# Autodesk Inventor assembly: Base-soporte
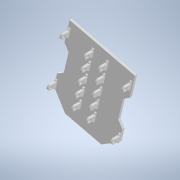
[picture p0: Inventor's stored thumbnail of the model, 180x180]
Saved by Autodesk Inventor 2021 (Build 250183000, 183)
## iProperties
Created: 2021-02-07
Part Number: Base-soporte
Document SubType Name: Assembly
Designer: rotje
Author: rotje
## Documents named in this file (5)
- C:\Users\rotje\Documents\Inventor\MSF\Base-soporte.iam
- C:\Users\rotje\Documents\Inventor\MSF\BaseCarro.ipt
- C:\Users\rotje\Documents\Inventor\MSF\sopoetellantas.ipt
- C:\Users\rotje\Documents\Inventor\MSF\soporte_para_engrane.ipt
- C:\Users\rotje\Documents\Inventor\MSF\din_912-m5x0_8-20-8_8.ipt
## Components (43 placed, 4 different names)
1. BaseCarro:1 — Insertar:1, Insertar:2, Insertar:3, Insertar:4, Insertar:5, Insertar:6, Insertar:7, Insertar:8, Insertar:9, Insertar:10, Insertar:11, Insertar:12, Insertar:13, Insertar:14, Insertar:15, Insertar:16, Insertar:17, Insertar:18, Insertar:19, Insertar:20, Insertar:21, Insertar:22, Insertar:23, Insertar:24, Insertar:25, Insertar:26, Insertar:27, Insertar:28
2. sopoetellantas:1 — Insertar:1, Insertar:2, Insertar:29, Insertar:30
3. sopoetellantas:2 — Insertar:7, Insertar:8, Insertar:35, Insertar:36
4. sopoetellantas:3 — Insertar:15, Insertar:16, Insertar:49, Insertar:50
5. sopoetellantas:4 — Insertar:9, Insertar:10, Insertar:51, Insertar:52
6. sopoetellantas:5 — Insertar:3, Insertar:4, Insertar:31, Insertar:32
7. sopoetellantas:6 — Insertar:5, Insertar:6, Insertar:33, Insertar:34
8. sopoetellantas:7 — Insertar:13, Insertar:14, Insertar:55, Insertar:56
9. sopoetellantas:8 — Insertar:11, Insertar:12, Insertar:53, Insertar:54
10. soporte_para_engrane:1 — Insertar:23, Insertar:24, Insertar:39, Insertar:40
11. soporte_para_engrane:2 — Insertar:25, Insertar:26, Insertar:41, Insertar:42
12. soporte_para_engrane:3 — Insertar:27, Insertar:28, Insertar:47, Insertar:48
13. soporte_para_engrane:4 — Insertar:17, Insertar:18, Insertar:37, Insertar:38
14. soporte_para_engrane:5 — Insertar:19, Insertar:20, Insertar:43, Insertar:44
15. soporte_para_engrane:6 — Insertar:21, Insertar:22, Insertar:45, Insertar:46
16. din_912-m5x0_8-20-8_8:1 — Insertar:29
17. din_912-m5x0_8-20-8_8:2 — Insertar:30
18. din_912-m5x0_8-20-8_8:3 — Insertar:32
19. din_912-m5x0_8-20-8_8:4 — Insertar:31
20. din_912-m5x0_8-20-8_8:5 — Insertar:33
21. din_912-m5x0_8-20-8_8:6 — Insertar:34
22. din_912-m5x0_8-20-8_8:7 — Insertar:35
23. din_912-m5x0_8-20-8_8:8 — Insertar:36
24. din_912-m5x0_8-20-8_8:9 — Insertar:39
25. din_912-m5x0_8-20-8_8:10 — Insertar:40
26. din_912-m5x0_8-20-8_8:11 — Insertar:41
27. din_912-m5x0_8-20-8_8:12 — Insertar:42
28. din_912-m5x0_8-20-8_8:13 — Insertar:47
29. din_912-m5x0_8-20-8_8:14 — Insertar:48
30. din_912-m5x0_8-20-8_8:15 — Insertar:49
31. din_912-m5x0_8-20-8_8:16 — Insertar:50
32. din_912-m5x0_8-20-8_8:17 — Insertar:53
33. din_912-m5x0_8-20-8_8:18 — Insertar:55
34. din_912-m5x0_8-20-8_8:19 — Insertar:54
35. din_912-m5x0_8-20-8_8:20 — Insertar:56
36. din_912-m5x0_8-20-8_8:21 — Insertar:51
37. din_912-m5x0_8-20-8_8:22 — Insertar:52
38. din_912-m5x0_8-20-8_8:23 — Insertar:37
39. din_912-m5x0_8-20-8_8:24 — Insertar:38
40. din_912-m5x0_8-20-8_8:25 — Insertar:43
41. din_912-m5x0_8-20-8_8:26 — Insertar:44
42. din_912-m5x0_8-20-8_8:27 — Insertar:45
43. din_912-m5x0_8-20-8_8:28 — Insertar:46
## Relationships (56: Insert 56)
- Insertar:1: BaseCarro:1 ↔ sopoetellantas:1
- Insertar:2: BaseCarro:1 ↔ sopoetellantas:1
- Insertar:3: BaseCarro:1 ↔ sopoetellantas:5
- Insertar:4: BaseCarro:1 ↔ sopoetellantas:5
- Insertar:5: BaseCarro:1 ↔ sopoetellantas:6
- Insertar:6: BaseCarro:1 ↔ sopoetellantas:6
- Insertar:7: BaseCarro:1 ↔ sopoetellantas:2
- Insertar:8: BaseCarro:1 ↔ sopoetellantas:2
- Insertar:9: BaseCarro:1 ↔ sopoetellantas:4
- Insertar:10: BaseCarro:1 ↔ sopoetellantas:4
- Insertar:11: BaseCarro:1 ↔ sopoetellantas:8
- Insertar:12: BaseCarro:1 ↔ sopoetellantas:8
- Insertar:13: BaseCarro:1 ↔ sopoetellantas:7
- Insertar:14: BaseCarro:1 ↔ sopoetellantas:7
- Insertar:15: BaseCarro:1 ↔ sopoetellantas:3
- Insertar:16: BaseCarro:1 ↔ sopoetellantas:3
- Insertar:17: BaseCarro:1 ↔ soporte_para_engrane:4
- Insertar:18: BaseCarro:1 ↔ soporte_para_engrane:4
- Insertar:19: BaseCarro:1 ↔ soporte_para_engrane:5
- Insertar:20: BaseCarro:1 ↔ soporte_para_engrane:5
- Insertar:21: BaseCarro:1 ↔ soporte_para_engrane:6
- Insertar:22: BaseCarro:1 ↔ soporte_para_engrane:6
- Insertar:23: BaseCarro:1 ↔ soporte_para_engrane:1
- Insertar:24: BaseCarro:1 ↔ soporte_para_engrane:1
- Insertar:25: BaseCarro:1 ↔ soporte_para_engrane:2
- Insertar:26: BaseCarro:1 ↔ soporte_para_engrane:2
- Insertar:27: BaseCarro:1 ↔ soporte_para_engrane:3
- Insertar:28: BaseCarro:1 ↔ soporte_para_engrane:3
- Insertar:29: sopoetellantas:1 ↔ din_912-m5x0_8-20-8_8:1
- Insertar:30: sopoetellantas:1 ↔ din_912-m5x0_8-20-8_8:2
- Insertar:31: sopoetellantas:5 ↔ din_912-m5x0_8-20-8_8:4
- Insertar:32: sopoetellantas:5 ↔ din_912-m5x0_8-20-8_8:3
- Insertar:33: sopoetellantas:6 ↔ din_912-m5x0_8-20-8_8:5
- Insertar:34: sopoetellantas:6 ↔ din_912-m5x0_8-20-8_8:6
- Insertar:35: sopoetellantas:2 ↔ din_912-m5x0_8-20-8_8:7
- Insertar:36: sopoetellantas:2 ↔ din_912-m5x0_8-20-8_8:8
- Insertar:37: soporte_para_engrane:4 ↔ din_912-m5x0_8-20-8_8:23
- Insertar:38: soporte_para_engrane:4 ↔ din_912-m5x0_8-20-8_8:24
- Insertar:39: soporte_para_engrane:1 ↔ din_912-m5x0_8-20-8_8:9
- Insertar:40: soporte_para_engrane:1 ↔ din_912-m5x0_8-20-8_8:10
- Insertar:41: soporte_para_engrane:2 ↔ din_912-m5x0_8-20-8_8:11
- Insertar:42: soporte_para_engrane:2 ↔ din_912-m5x0_8-20-8_8:12
- Insertar:43: soporte_para_engrane:5 ↔ din_912-m5x0_8-20-8_8:25
- Insertar:44: soporte_para_engrane:5 ↔ din_912-m5x0_8-20-8_8:26
- Insertar:45: soporte_para_engrane:6 ↔ din_912-m5x0_8-20-8_8:27
- Insertar:46: soporte_para_engrane:6 ↔ din_912-m5x0_8-20-8_8:28
- Insertar:47: soporte_para_engrane:3 ↔ din_912-m5x0_8-20-8_8:13
- Insertar:48: soporte_para_engrane:3 ↔ din_912-m5x0_8-20-8_8:14
- Insertar:49: sopoetellantas:3 ↔ din_912-m5x0_8-20-8_8:15
- Insertar:50: sopoetellantas:3 ↔ din_912-m5x0_8-20-8_8:16
- Insertar:51: sopoetellantas:4 ↔ din_912-m5x0_8-20-8_8:21
- Insertar:52: sopoetellantas:4 ↔ din_912-m5x0_8-20-8_8:22
- Insertar:53: sopoetellantas:8 ↔ din_912-m5x0_8-20-8_8:17
- Insertar:54: sopoetellantas:8 ↔ din_912-m5x0_8-20-8_8:19
- Insertar:55: sopoetellantas:7 ↔ din_912-m5x0_8-20-8_8:18
- Insertar:56: sopoetellantas:7 ↔ din_912-m5x0_8-20-8_8:20
